# Autodesk Inventor assembly: Ball_Bearing_Holder_Assembly
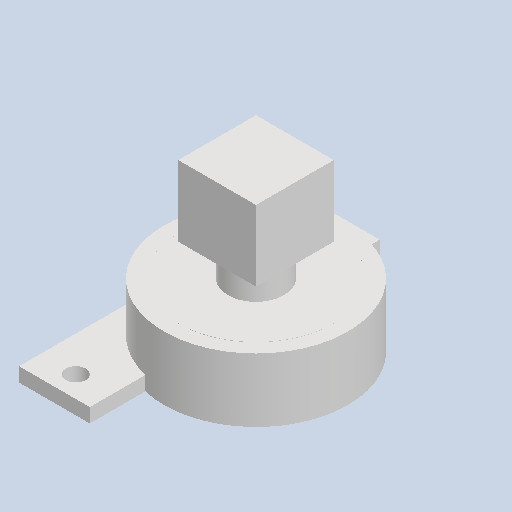
[picture p0: Inventor's stored thumbnail of the model, 512x512]
Saved by Autodesk Inventor 2022 (Build 260153000, 153)
## iProperties
Created: 2023-03-18
Part Number: Ball_Bearing_Holder_Assembly
Document SubType Name: Assembly
Designer: zarek
Author: zarek
## Documents named in this file (4)
- C:\Users\zarek\OneDrive\Desktop\Random New Stuff\SPB\Ball_Bearing_Holder_Assembly.iam
- C:\Users\zarek\OneDrive\Desktop\Random New Stuff\SPB\Ball_Bearing_Holder.ipt
- C:\Users\zarek\OneDrive\Desktop\Random New Stuff\SPB\Ball_Bearing_Mock_8_22_7mm.ipt
- C:\Users\zarek\OneDrive\Desktop\Random New Stuff\SPB\Motor_Key_Bearing_2.ipt
## Components (3 placed, 3 different names)
1. Ball_Bearing_Holder:1 — Mate:1
2. Ball_Bearing_Mock_8_22_7mm:1 — Mate:1, Mate:2
3. Motor_Key_Bearing_2:1 — Mate:2
## Relationships (2: Mate 2)
- Mate:1: Ball_Bearing_Holder:1 ↔ Ball_Bearing_Mock_8_22_7mm:1
- Mate:2: Ball_Bearing_Mock_8_22_7mm:1 ↔ Motor_Key_Bearing_2:1
